# Autodesk Inventor assembly: Avi Bay Start
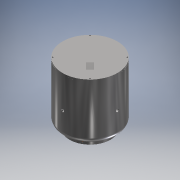
[picture p0: Inventor's stored thumbnail of the model, 180x180]
Saved by Autodesk Inventor 2017 (Build 210142000, 142)
## iProperties
Created: 2016-11-08
Part Number: Avi Bay Start
Document SubType Name: Assembly
Designer: mnweir
Author: mnweir
## Documents named in this file (4)
- \\acsnfs4.ucsd.edu\CifsHomes\690\mnweir\Avi Bay Start.iam
- \\acsnfs4.ucsd.edu\CifsHomes\690\mnweir\Avi Bay Steel.ipt
- \\acsnfs4.ucsd.edu\CifsHomes\690\mnweir\Avi Bay phenolic.ipt
- \\acsnfs4.ucsd.edu\CifsHomes\690\mnweir\Avi Bay Lid.ipt
## Components (3 placed, 3 different names)
1. Avi Bay Steel:1 — Cylindrical:1, Rotational:1
2. Avi Bay phenolic:1 — Cylindrical:1
3. Avi Bay Lid:1 — Rotational:1
## Relationships (2: CylindricalJoint 1, RevoluteJoint 1)
- Cylindrical:1: Avi Bay Steel:1 ↔ Avi Bay phenolic:1
- Rotational:1 [RevoluteJoint]: Avi Bay Steel:1 ↔ Avi Bay Lid:1
